# Autodesk Inventor assembly: TCRT5000
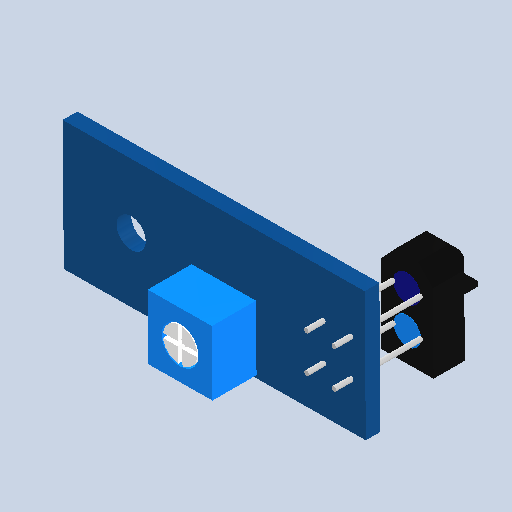
[picture p0: Inventor's stored thumbnail of the model, 512x512]
Saved by Autodesk Inventor 2022 (Build 260153000, 153)
## iProperties
Created: 2025-01-12
Part Number: TCRT5000
Description: STEP AP214
Document SubType Name: Assembly
Designer: Admin
Preprocessor: Spatial InterOp 3D
Title: TCRT5000.stp
Revision Number: NONE
## Documents named in this file (6)
- G:\abuyz lkz vfibyrb\TCRT5000.iam
- G:\abuyz lkz vfibyrb\TCRT5000.ipt
- G:\abuyz lkz vfibyrb\Board Geometry.ipt
- G:\abuyz lkz vfibyrb\pins.ipt
- G:\abuyz lkz vfibyrb\leds2 Geometry.ipt
- G:\abuyz lkz vfibyrb\pot Geometry.ipt
## Components (5 placed, 5 different names)
1. TCRT5000 — Заподлицо:2, Заподлицо:3, Заподлицо:4
2. Board Geometry — Заподлицо:2, Заподлицо:3, Заподлицо:4, Совмещение:2, Заподлицо:5, Заподлицо:6
3. pins
4. leds2 Geometry
5. pot Geometry — Совмещение:2, Заподлицо:5, Заподлицо:6
## Relationships (9: Flush 6, Mate 2, Insert 1)
- [Flush]: TCRT5000 ↔ leds2 Geometry
- [Insert]: TCRT5000 ↔ leds2 Geometry
- [Mate]: TCRT5000 ↔ leds2 Geometry
- Заподлицо:2 [Flush] (-10 mm): TCRT5000 ↔ Board Geometry
- Заподлицо:3 [Flush] (1.9 mm): TCRT5000 ↔ Board Geometry
- Заподлицо:4 [Flush] (-0.2 mm): TCRT5000 ↔ Board Geometry
- Совмещение:2 [Mate]: Board Geometry ↔ pot Geometry
- Заподлицо:5 [Flush] (0.3 mm): Board Geometry ↔ pot Geometry
- Заподлицо:6 [Flush] (14 mm): Board Geometry ↔ pot Geometry
